# Autodesk Inventor assembly: 全体
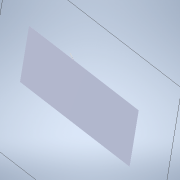
[picture p0: Inventor's stored thumbnail of the model, 180x180]
Saved by Autodesk Inventor 2020.3 (Build 243373000, 373)
## iProperties
Created: 2020-05-31
Part Number: 全体
Document SubType Name: Assembly
Designer: totot
Author: totot
## Documents named in this file (4)
- D:\mysvn\ロボコン\キャチロボ\キャチロボ設計図\全体.iam
- D:\mysvn\ロボコン\キャチロボ\キャチロボ設計図\フィールド\フィールド.iam
- D:\mysvn\ロボコン\キャチロボ\キャチロボ設計図\ロボット\ロボット.iam
- D:\mysvn\ロボコン\キャチロボ\キャチロボ設計図\フィールド\[N.ipt
## Components (3 placed, 3 different names)
1. フィールド:1 [sub-assembly] — 挿入:2, 挿入:3, メイト:1
2. ロボット:1 [sub-assembly] — 挿入:2, 挿入:3
3. [N:1 — メイト:1
## Relationships (3: Insert 2, Mate 1)
- 挿入:2 [Insert]: フィールド:1 ↔ ロボット:1
- 挿入:3 [Insert]: フィールド:1 ↔ ロボット:1
- メイト:1 [Mate]: フィールド:1 ↔ [N:1
